# Autodesk Inventor assembly: ASY TZS 0940 FDS Top elbow
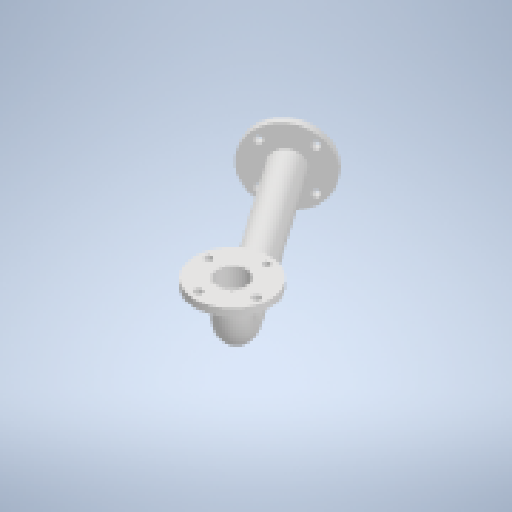
[picture p0: Inventor's stored thumbnail of the model, 512x512]
Saved by Autodesk Inventor 2025 (Build 290162010, 162A)
## iProperties
Created: 2025-07-10
Part Number: ASY TZS 0940 FDS Top elbow
Document SubType Name: Assembly
Designer: user
Author: user
## Documents named in this file (5)
- C:\Users\pokla\Documents\Inventor\TZS-Tazovskiy\Filter D940\ASY TZS 0940 FDS Top elbow.iam
- C:\Users\pokla\Documents\Inventor\TZS-Tazovskiy\Filter D940\TZS 0942 FDS  tube 1.ipt
- C:\Users\pokla\Documents\Inventor\TZS-Tazovskiy\Filter D940\TZS 0941 FDS tube 1.ipt
- C:\Users\pokla\Documents\Inventor\Content Center Files\R2025\en-US\JIS B 2312 90 (2)\JIS B 2312 90 Deg Long Elbow Steel 65A x Sch 40.ipt
- C:\Users\pokla\Documents\Inventor\Content Center Files\R2025\en-US\DIN 2576 PN 10(2)\DIN 2576 Slip-On Flange for Welding Series 1 (ISO) - PN 10 65 x 76.1.ipt
## Components (5 placed, 4 different names)
1. TZS 0941 FDS tube 1.ipt:1 — Rigid:11
2. JIS B 2312 90 Deg Long Elbow Steel 65A x Sch 40.ipt:1
3. TZS 0942 FDS  tube 1.ipt:1 — Rigid:10
4. DIN 2576 Slip-On Flange for Welding Series 1 (ISO) - PN 10 65 x 76.1:4 — Rigid:10
5. DIN 2576 Slip-On Flange for Welding Series 1 (ISO) - PN 10 65 x 76.1:5 — Rigid:11
## Relationships (4: WeldJoint 4)
- [WeldJoint]: TZS 0941 FDS tube 1.ipt:1 ↔ JIS B 2312 90 Deg Long Elbow Steel 65A x Sch 40.ipt:1
- [WeldJoint]: JIS B 2312 90 Deg Long Elbow Steel 65A x Sch 40.ipt:1 ↔ TZS 0942 FDS  tube 1.ipt:1
- Rigid:10 [WeldJoint]: TZS 0942 FDS  tube 1.ipt:1 ↔ DIN 2576 Slip-On Flange for Welding Series 1 (ISO) - PN 10 65 x 76.1:4
- Rigid:11 [WeldJoint]: TZS 0941 FDS tube 1.ipt:1 ↔ DIN 2576 Slip-On Flange for Welding Series 1 (ISO) - PN 10 65 x 76.1:5
